# Autodesk Inventor assembly: Stock Dicoeasy Assembly-rebuild take 3
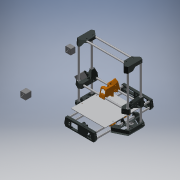
[picture p0: Inventor's stored thumbnail of the model, 180x180]
Saved by Autodesk Inventor 2017 (Build 210142000, 142)
## iProperties
Created: 2017-03-10
Part Number: Stock Dicoeasy Assembly-rebuild take 3
Document SubType Name: Assembly
Designer: gilef
Author: gilef
## Documents named in this file (20)
- C:\Users\gilef\Documents\Inventor\DiscoEasy200\Stock Dicoeasy Assembly-rebuild take 3.iam
- C:\Users\gilef\Documents\Inventor\DiscoEasy200\Original Plate Mount.ipt
- C:\Users\gilef\Documents\Inventor\DiscoEasy200\Original Rear Left Plate Mount.ipt
- C:\Users\gilef\Documents\Inventor\DiscoEasy200\Original Rear Right Plate Mount.ipt
- C:\Users\gilef\Documents\Inventor\DiscoEasy200\Converted LM8UU Linear Bearing.ipt
- C:\Users\gilef\Documents\Inventor\DiscoEasy200\Stock Build Plate.ipt
- C:\Users\gilef\Documents\Inventor\Content Center Files\R2017\en-US\AS 1427(07)\AS 1427 - M3 x 10(6) II.ipt
- C:\Users\gilef\Documents\Inventor\Content Center Files\R2017\en-US\ANSI B18.16.3M(2)\ANSI B18.16.3M - Property Class 5 and 10 - Metric M3 x 0.5 Metal Type.ipt
- C:\Users\gilef\Documents\Inventor\DiscoEasy200\Stock Front Plate.ipt
- C:\Users\gilef\Documents\Inventor\DiscoEasy200\Stock Back Plate.ipt
- C:\Users\gilef\Documents\Inventor\DiscoEasy200\Long Metal Rod.ipt
- C:\Users\gilef\Documents\Inventor\DiscoEasy200\Short Metal Rod.ipt
- C:\Users\gilef\Documents\Inventor\DiscoEasy200\Original Printer Base.ipt
- C:\Users\gilef\Documents\Inventor\DiscoEasy200\Stock Left Top.ipt
- C:\Users\gilef\Documents\Inventor\DiscoEasy200\Stock Top Right.ipt
- C:\Users\gilef\Documents\Inventor\DiscoEasy200\Stock X Axis Left (Extruder).ipt
- C:\Users\gilef\Documents\Inventor\DiscoEasy200\Stock X Axis Right.ipt
- C:\Users\gilef\Documents\Inventor\DiscoEasy200\Stock Extruder Head.ipt
- C:\Users\gilef\Documents\Inventor\DiscoEasy200\XY Stepper Motor.ipt
- C:\Users\gilef\Documents\Inventor\DiscoEasy200\Z Stepper Motor.ipt
## Components (48 placed, 19 different names)
1. Original Plate Mount:1 — Flush:2, Mate:1, Flush:3, Mate:2, Mate:7, Mate:8, Mate:9, Mate:10, Mate:11, Insert:7, Angle:3, Insert:10, Angle:4
2. Original Rear Right Plate Mount:1 — Flush:2, Mate:1, Mate:3, Mate:4, Flush:4, Insert:9, Angle:1
3. Original Rear Left Plate Mount:1 — Flush:3, Mate:2, Mate:5, Mate:6, Flush:4, Insert:1, Insert:6, Angle:2
4. Converted LM8UU Linear Bearing:1 — Mate:7, Mate:8, Mate:15
5. Converted LM8UU Linear Bearing:2 — Mate:3, Mate:4, Mate:12
6. Converted LM8UU Linear Bearing:3 — Mate:9, Mate:10, Mate:14
7. Converted LM8UU Linear Bearing:4 — Mate:5, Mate:6, Mate:13
8. Stock Build Plate:1 — Insert:1, Mate:11, Insert:2, Insert:3, Insert:4, Insert:5
9. AS 1427 Z - Metric M3 x 10:1 — Insert:2
10. AS 1427 Z - Metric M3 x 10:2 — Insert:3
11. AS 1427 Z - Metric M3 x 10:3 — Insert:4
12. AS 1427 Z - Metric M3 x 10:4 — Insert:5
13. Prevailing Torque Type Hex Nut - Steel Metric Property Class 5 and 10 - Metric M3 x 0.5 Metal Type:1 — Insert:10, Angle:4
14. Prevailing Torque Type Hex Nut - Steel Metric Property Class 5 and 10 - Metric M3 x 0.5 Metal Type:2 — Insert:9, Angle:1
15. Prevailing Torque Type Hex Nut - Steel Metric Property Class 5 and 10 - Metric M3 x 0.5 Metal Type:3 — Insert:7, Angle:3
16. Prevailing Torque Type Hex Nut - Steel Metric Property Class 5 and 10 - Metric M3 x 0.5 Metal Type:4 — Insert:6, Angle:2
17. Stock Front Plate:1 — Mate:14, Mate:15, Flush:5, Insert:14, Insert:15, Insert:16, Insert:17, Mate:71
18. Stock Back Plate:1 — Mate:12, Mate:13, Insert:13
19. Long Metal Rod:1 — Insert:16
20. Long Metal Rod:2 — Insert:15
21. Long Metal Rod:3 — Insert:17
22. Long Metal Rod:4 — Insert:13, Insert:14, Mate:54
23. Short Metal Rod:1 — Insert:18, Insert:19
24. Original Printer Base:1 — Flush:6, Insert:18, Mate:54, Insert:20, Insert:21
25. Original Printer Base:2 — Flush:5, Flush:6, Mate:30, Mate:31, Mate:34, Mate:35, Insert:19, Mate:71, Mate:76, Mate:77, Angle:5
26. Long Metal Rod:5 — Mate:30, Mate:35, Mate:50, Mate:58
27. Long Metal Rod:6 — Mate:31, Mate:34, Mate:51, Mate:57
28. Long Metal Rod:7 — Insert:20, Insert:22, Mate:55
29. Long Metal Rod:8 — Insert:21, Insert:23, Mate:56
30. Stock Left Top:1 — Insert:26, Insert:27
31. Stock Top Right:1 — Insert:22, Insert:23, Insert:24, Insert:25
32. Short Metal Rod:2 — Insert:24, Insert:26
33. Short Metal Rod:3 — Insert:25, Insert:27
34. Stock X Axis Left (Extruder):1 — Insert:11, Insert:12, Mate:60, Mate:61, Mate:62, Mate:63, Flush:7, Mate:73, Mate:74, Mate:75
35. Stock X Axis Right:1 — Mate:50, Mate:51, Mate:59, Mate:64, Flush:7
36. Short Metal Rod:4 — Insert:11, Mate:69
37. Short Metal Rod:5 — Insert:12, Mate:70
38. Converted LM8UU Linear Bearing:5 — Mate:58, Mate:64
39. Converted LM8UU Linear Bearing:6 — Mate:57, Mate:59
40. Converted LM8UU Linear Bearing:7 — Mate:55, Mate:61, Mate:62
41. Converted LM8UU Linear Bearing:8 — Mate:56, Mate:60, Mate:63
42. Stock Extruder Head:1 — Mate:65, Mate:66, Mate:67, Mate:68
43. Converted LM8UU Linear Bearing:9 — Mate:65, Mate:68, Mate:70
44. Converted LM8UU Linear Bearing:10 — Mate:66, Mate:67, Mate:69
45. XY Stepper Motor:1 — Mate:73, Mate:74, Mate:75
46. Z Stepper Motor:1 — Mate:76, Mate:77, Angle:5
47. XY Stepper Motor:2
48. Z Stepper Motor:2
## Relationships (81: Mate 44, Insert 26, Flush 6, Angle 5)
- Flush:2: Original Plate Mount:1 ↔ Original Rear Right Plate Mount:1
- Mate:1: Original Plate Mount:1 ↔ Original Rear Right Plate Mount:1
- Flush:3: Original Plate Mount:1 ↔ Original Rear Left Plate Mount:1
- Mate:2: Original Plate Mount:1 ↔ Original Rear Left Plate Mount:1
- Mate:3: Original Rear Right Plate Mount:1 ↔ Converted LM8UU Linear Bearing:2
- Mate:4: Original Rear Right Plate Mount:1 ↔ Converted LM8UU Linear Bearing:2
- Mate:5: Original Rear Left Plate Mount:1 ↔ Converted LM8UU Linear Bearing:4
- Mate:6: Original Rear Left Plate Mount:1 ↔ Converted LM8UU Linear Bearing:4
- Mate:7: Original Plate Mount:1 ↔ Converted LM8UU Linear Bearing:1
- Mate:8: Original Plate Mount:1 ↔ Converted LM8UU Linear Bearing:1
- Mate:9: Original Plate Mount:1 ↔ Converted LM8UU Linear Bearing:3
- Mate:10: Original Plate Mount:1 ↔ Converted LM8UU Linear Bearing:3
- Flush:4: Original Rear Right Plate Mount:1 ↔ Original Rear Left Plate Mount:1
- Insert:1: Original Rear Left Plate Mount:1 ↔ Stock Build Plate:1
- Mate:11: Original Plate Mount:1 ↔ Stock Build Plate:1
- Insert:2: Stock Build Plate:1 ↔ AS 1427 Z - Metric M3 x 10:1
- Insert:3: Stock Build Plate:1 ↔ AS 1427 Z - Metric M3 x 10:2
- Insert:4: Stock Build Plate:1 ↔ AS 1427 Z - Metric M3 x 10:3
- Insert:5: Stock Build Plate:1 ↔ AS 1427 Z - Metric M3 x 10:4
- Insert:6: Original Rear Left Plate Mount:1 ↔ Prevailing Torque Type Hex Nut - Steel Metric Property Class 5 and 10 - Metric M3 x 0.5 Metal Type:4
- Insert:7: Original Plate Mount:1 ↔ Prevailing Torque Type Hex Nut - Steel Metric Property Class 5 and 10 - Metric M3 x 0.5 Metal Type:3
- Insert:9: Original Rear Right Plate Mount:1 ↔ Prevailing Torque Type Hex Nut - Steel Metric Property Class 5 and 10 - Metric M3 x 0.5 Metal Type:2
- Angle:1 (0 deg): Original Rear Right Plate Mount:1 ↔ Prevailing Torque Type Hex Nut - Steel Metric Property Class 5 and 10 - Metric M3 x 0.5 Metal Type:2
- Angle:2 (0 deg): Original Rear Left Plate Mount:1 ↔ Prevailing Torque Type Hex Nut - Steel Metric Property Class 5 and 10 - Metric M3 x 0.5 Metal Type:4
- Angle:3 (0 deg): Original Plate Mount:1 ↔ Prevailing Torque Type Hex Nut - Steel Metric Property Class 5 and 10 - Metric M3 x 0.5 Metal Type:3
- Insert:10: Original Plate Mount:1 ↔ Prevailing Torque Type Hex Nut - Steel Metric Property Class 5 and 10 - Metric M3 x 0.5 Metal Type:1
- Angle:4 (0 deg): Original Plate Mount:1 ↔ Prevailing Torque Type Hex Nut - Steel Metric Property Class 5 and 10 - Metric M3 x 0.5 Metal Type:1
- Mate:12: Converted LM8UU Linear Bearing:2 ↔ Stock Back Plate:1
- Mate:13: Converted LM8UU Linear Bearing:4 ↔ Stock Back Plate:1
- Mate:14: Converted LM8UU Linear Bearing:3 ↔ Stock Front Plate:1
- Mate:15: Converted LM8UU Linear Bearing:1 ↔ Stock Front Plate:1
- Flush:5: Stock Front Plate:1 ↔ Original Printer Base:2
- Flush:6: Original Printer Base:1 ↔ Original Printer Base:2
- Mate:30: Original Printer Base:2 ↔ Long Metal Rod:5
- Mate:31: Original Printer Base:2 ↔ Long Metal Rod:6
- Mate:34: Original Printer Base:2 ↔ Long Metal Rod:6
- Mate:35: Original Printer Base:2 ↔ Long Metal Rod:5
- Mate:50: Long Metal Rod:5 ↔ Stock X Axis Right:1
- Mate:51: Long Metal Rod:6 ↔ Stock X Axis Right:1
- Insert:11: Stock X Axis Left (Extruder):1 ↔ Short Metal Rod:4
- Insert:12: Stock X Axis Left (Extruder):1 ↔ Short Metal Rod:5
- Insert:13: Stock Back Plate:1 ↔ Long Metal Rod:4
- Insert:14: Stock Front Plate:1 ↔ Long Metal Rod:4
- Insert:15: Stock Front Plate:1 ↔ Long Metal Rod:2
- Insert:16: Stock Front Plate:1 ↔ Long Metal Rod:1
- Insert:17: Stock Front Plate:1 ↔ Long Metal Rod:3
- Insert:18: Short Metal Rod:1 ↔ Original Printer Base:1
- Insert:19: Short Metal Rod:1 ↔ Original Printer Base:2
- Mate:54: Long Metal Rod:4 ↔ Original Printer Base:1
- Insert:20: Original Printer Base:1 ↔ Long Metal Rod:7
- Insert:21: Original Printer Base:1 ↔ Long Metal Rod:8
- Insert:22: Long Metal Rod:7 ↔ Stock Top Right:1
- Insert:23: Long Metal Rod:8 ↔ Stock Top Right:1
- Insert:24: Stock Top Right:1 ↔ Short Metal Rod:2
- Insert:25: Stock Top Right:1 ↔ Short Metal Rod:3
- Insert:26: Stock Left Top:1 ↔ Short Metal Rod:2
- Insert:27: Stock Left Top:1 ↔ Short Metal Rod:3
- Mate:55: Long Metal Rod:7 ↔ Converted LM8UU Linear Bearing:7
- Mate:56: Long Metal Rod:8 ↔ Converted LM8UU Linear Bearing:8
- Mate:57: Long Metal Rod:6 ↔ Converted LM8UU Linear Bearing:6
- Mate:58: Long Metal Rod:5 ↔ Converted LM8UU Linear Bearing:5
- Mate:59: Stock X Axis Right:1 ↔ Converted LM8UU Linear Bearing:6
- Mate:60: Stock X Axis Left (Extruder):1 ↔ Converted LM8UU Linear Bearing:8
- Mate:61: Stock X Axis Left (Extruder):1 ↔ Converted LM8UU Linear Bearing:7
- Mate:62: Stock X Axis Left (Extruder):1 ↔ Converted LM8UU Linear Bearing:7
- Mate:63: Stock X Axis Left (Extruder):1 ↔ Converted LM8UU Linear Bearing:8
- Mate:64: Stock X Axis Right:1 ↔ Converted LM8UU Linear Bearing:5
- Flush:7: Stock X Axis Left (Extruder):1 ↔ Stock X Axis Right:1
- Mate:65: Stock Extruder Head:1 ↔ Converted LM8UU Linear Bearing:9
- Mate:66: Stock Extruder Head:1 ↔ Converted LM8UU Linear Bearing:10
- Mate:67 (1.2 mm): Stock Extruder Head:1 ↔ Converted LM8UU Linear Bearing:10
- Mate:68 (1.2 mm): Stock Extruder Head:1 ↔ Converted LM8UU Linear Bearing:9
- Mate:69: Short Metal Rod:4 ↔ Converted LM8UU Linear Bearing:10
- Mate:70: Short Metal Rod:5 ↔ Converted LM8UU Linear Bearing:9
- Mate:71 (170 mm): Stock Front Plate:1 ↔ Original Printer Base:2
- Mate:73: Stock X Axis Left (Extruder):1 ↔ XY Stepper Motor:1
- Mate:74: Stock X Axis Left (Extruder):1 ↔ XY Stepper Motor:1
- Mate:75: Stock X Axis Left (Extruder):1 ↔ XY Stepper Motor:1
- Mate:76: Original Printer Base:2 ↔ Z Stepper Motor:1
- Mate:77: Original Printer Base:2 ↔ Z Stepper Motor:1
- Angle:5 (45 deg): Original Printer Base:2 ↔ Z Stepper Motor:1
